# Autodesk Inventor assembly: EnsambleEngrane
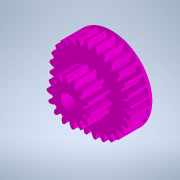
[picture p0: Inventor's stored thumbnail of the model, 180x180]
Saved by Autodesk Inventor 2022 (Build 260153000, 153)
## iProperties
Created: 2022-02-25
Part Number: EnsambleEngrane
Document SubType Name: Assembly
Designer: hurta
Author: hurta
## Documents named in this file (3)
- C:\Users\hurta\Documents\Universidad\NovenoSemestre\MiniProyecto1\MiniProyecto1\Diseno_Mecanico_Inventor\Transmision_Potencia\TrenEngrane_SegundaEtapa.iam
- C:\Users\hurta\Documents\Universidad\NovenoSemestre\MiniProyecto1\MiniProyecto1\Diseno_Mecanico_Inventor\Transmision_Potencia\Engrane28Dientes.ipt
- C:\Users\hurta\Documents\Universidad\NovenoSemestre\MiniProyecto1\MiniProyecto1\Diseno_Mecanico_Inventor\Transmision_Potencia\Engrane14Dientes.ipt
## Components (2 placed, 2 different names)
1. Engrane28Dientes:1 — Mate:1, Mate:2
2. Engrane14Dientes:1 — Mate:1, Mate:2
## Relationships (2: Mate 2)
- Mate:1: Engrane28Dientes:1 ↔ Engrane14Dientes:1
- Mate:2: Engrane28Dientes:1 ↔ Engrane14Dientes:1
